# Autodesk Inventor assembly: FE-00035-02
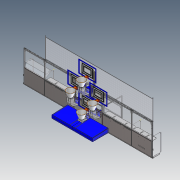
[picture p0: Inventor's stored thumbnail of the model, 180x180]
Saved by Autodesk Inventor 2012 (Build 160160000, 160)
## iProperties
Created: 2010-11-28
Part Number: FE-00035-02
Document SubType Name: Assembly
Designer: dfoster
Description: End Panel Sub-Assembly
Title: End Panel Sub-Assembly
Author: dfoster
## Documents named in this file (24)
- C:\Data Folder\FRC 2012 Field\Components\FE-00035-02.iam
- C:\Data Folder\FRC 2012 Field\Components\FE-00004.iam
- C:\Data Folder\FRC 2012 Field\Components\FE-00001.iam
- C:\Data Folder\FRC 2012 Field\Components\FE-00002-11.iam
- C:\Data Folder\FRC 2012 Field\Components\FE-00002-12.iam
- C:\Data Folder\FRC 2012 Field\Components\FE-00012.ipt
- C:\Data Folder\FRC 2012 Field\Components\GE-11041r.iam
- C:\Data Folder\FRC 2012 Field\Components\GE-11041L.iam
- C:\Data Folder\FRC 2012 Field\Components\GE-09031.iam
- C:\Data Folder\FRC 2012 Field\Components\FE-00007.iam
- C:\Data Folder\FRC 2012 Field\Components\GE-12096.iam
- C:\Data Folder\FRC 2012 Field\Components\GE-12051.ipt
- C:\Data Folder\FRC 2012 Field\Components\GE-12055.ipt
- C:\Data Folder\FRC 2012 Field\Components\GE-12053.iam
- C:\Data Folder\FRC 2012 Field\Components\GE-12057.iam
- C:\Data Folder\FRC 2012 Field\Components\GE-12057_left.iam
- C:\Data Folder\FRC 2012 Field\Components\GE-12056.ipt
- C:\Data Folder\FRC 2012 Field\Components\GE-12078.iam
- C:\Data Folder\FRC 2012 Field\Components\GE-12091.iam
- C:\Data Folder\FRC 2012 Field\Components\GE-12060.ipt
- C:\Data Folder\FRC 2012 Field\Components\GE-12104.ipt
- C:\Data Folder\FRC 2012 Field\Components\HW-00005.0005.ipt
- C:\Data Folder\FRC 2012 Field\Components\HW-00063.ipt
- C:\Data Folder\FRC 2012 Field\Components\HW-00002.ipt
## Components (38 placed, 23 different names)
1. GE-09031:1 [sub-assembly] — Flush:31, Flush:32, Tangent:10, Tangent:15
2. GE-09031:2 [sub-assembly] — Flush:29, Flush:30, Tangent:9, Tangent:16
3. GE-11041r:1 [sub-assembly] — Flush:17, Flush:18, Flush:21, Flush:22, Mate:12, Mate:23, Mate:28, Mate:30, Mate:31, Flush:44
4. GE-11041L:1 [sub-assembly] — Flush:19, Flush:20, Flush:23, Flush:24, Mate:13, Mate:26, Mate:48, Mate:49, Flush:56
5. FE-00002-11:1 [sub-assembly] — Flush:21, Flush:22, Mate:12, Tangent:15, Mate:34, Mate:35, Flush:46, Tangent:19
6. FE-00012:3 — Mate:20, Mate:21, Flush:37, Flush:43, Mate:29
7. FE-00012:1 — Mate:15, Mate:16, Flush:33, Flush:41, Flush:42, Mate:27
8. FE-00002-12:1 [sub-assembly] — Flush:23, Flush:24, Mate:13, Tangent:16
9. FE-00001:3 [sub-assembly] — Mate:7, Flush:13, Flush:14, Flush:17, Tangent:10, Tangent:14, Mate:23, Mate:24
10. FE-00001:4 [sub-assembly] — Flush:9, Mate:5, Flush:10, Flush:19, Tangent:3, Mate:14, Tangent:6, Tangent:9, Mate:26, Mate:36, Mate:37, Flush:47, Tangent:20
11. FE-00004:3 [sub-assembly] — Mate:7, Flush:13, Flush:14, Flush:18, Mate:20, Mate:21, Flush:35, Flush:36, Mate:22, Flush:37
12. FE-00004:2 [sub-assembly] — Flush:9, Mate:5, Flush:10, Flush:20, Mate:15, Mate:16, Flush:33, Flush:38, Mate:25, Flush:39
13. FE-00007:1 [sub-assembly] — Tangent:3, Mate:14, Tangent:6, Flush:29, Flush:30, Flush:40
14. FE-00007:3 [sub-assembly] — Flush:31, Flush:32, Tangent:14, Tangent:17, Mate:24, Flush:40
15. GE-12096:1 [sub-assembly] — Flush:34, Flush:35, Flush:36, Mate:22, Tangent:17, Flush:38, Mate:25, Flush:39, Mate:43, Mate:44, Mate:45, Mate:46, Mate:47, Insert:1, Insert:2, Insert:3, Insert:4
16. GE-12051:1 — Flush:41, Flush:42, Mate:27
17. GE-12055:1 — Flush:43, Mate:28, Mate:29
18. GE-12053:1 [sub-assembly] — Mate:30, Mate:31, Flush:44, Insert:5, Insert:6, Mate:52, Mate:53
19. GE-12060:1 — Mate:48, Mate:49, Flush:56
20. GE-12057:1 [sub-assembly] — Mate:36, Mate:37, Flush:47, Mate:39
21. GE-12057_left:1 [sub-assembly] — Mate:34, Mate:35, Flush:46, Mate:38
22. GE-12056:1 — Mate:38, Tangent:19
23. GE-12056:2 — Mate:39, Tangent:20
24. GE-12104:1
25. GE-12078:1 [sub-assembly] — Mate:43, Mate:44, Flush:55
26. GE-12091:1 [sub-assembly] — Flush:55, Mate:45, Mate:46, Mate:47
27. HW-00005.0005:1 — Insert:4
28. HW-00005.0005:2 — Insert:3
29. HW-00005.0005:3 — Insert:2
30. HW-00005.0005:4 — Insert:1
31. HW-00063:1 — Insert:5, Mate:50
32. HW-00063:2 — Insert:6, Mate:51
33. HW-00002:1 — Mate:50, Mate:52
34. HW-00002:2 — Mate:51, Mate:53
35. HW-00063:3
36. HW-00063:4
37. HW-00002:3
38. HW-00002:4
## Component patterns: (2 elements, first: HW-00063:1 + HW-00063:2 + HW-00002:1 + HW-00002:2)
## Relationships (88: Mate 39, Flush 33, Tangent 10, Insert 6)
- Flush:9: FE-00001:4 ↔ FE-00004:2
- Mate:5 (3.175 mm): FE-00001:4 ↔ FE-00004:2
- Flush:10: FE-00001:4 ↔ FE-00004:2
- Mate:7 (3.175 mm): FE-00001:3 ↔ FE-00004:3
- Flush:13: FE-00001:3 ↔ FE-00004:3
- Flush:14: FE-00001:3 ↔ FE-00004:3
- Flush:17: GE-11041r:1 ↔ FE-00001:3
- Flush:18: GE-11041r:1 ↔ FE-00004:3
- Flush:19: GE-11041L:1 ↔ FE-00001:4
- Flush:20: GE-11041L:1 ↔ FE-00004:2
- Flush:21: GE-11041r:1 ↔ FE-00002-11:1
- Flush:22: GE-11041r:1 ↔ FE-00002-11:1
- Mate:12 (22.225 mm): GE-11041r:1 ↔ FE-00002-11:1
- Flush:23: GE-11041L:1 ↔ FE-00002-12:1
- Flush:24: GE-11041L:1 ↔ FE-00002-12:1
- Mate:13 (22.225 mm): GE-11041L:1 ↔ FE-00002-12:1
- Tangent:3 (0.7874 mm): FE-00001:4 ↔ FE-00007:1
- Mate:14: FE-00001:4 ↔ FE-00007:1
- Tangent:6: FE-00001:4 ↔ FE-00007:1
- Flush:29: GE-09031:2 ↔ FE-00007:1
- Flush:30: GE-09031:2 ↔ FE-00007:1
- Tangent:9: GE-09031:2 ↔ FE-00001:4
- Flush:31: GE-09031:1 ↔ FE-00007:3
- Flush:32: GE-09031:1 ↔ FE-00007:3
- Tangent:10: GE-09031:1 ↔ FE-00001:3
- Mate:15: FE-00012:1 ↔ FE-00004:2
- Mate:16: FE-00012:1 ↔ FE-00004:2
- Flush:33: FE-00012:1 ↔ FE-00004:2
- Mate:20: FE-00012:3 ↔ FE-00004:3
- Mate:21: FE-00012:3 ↔ FE-00004:3
- Tangent:14 (0.7874 mm): FE-00001:3 ↔ FE-00007:3
- Tangent:15: GE-09031:1 ↔ FE-00002-11:1
- Tangent:16: GE-09031:2 ↔ FE-00002-12:1
- Flush:34: GE-12096:1
- Flush:35: FE-00004:3 ↔ GE-12096:1
- Flush:36: FE-00004:3 ↔ GE-12096:1
- Mate:22 (3.175 mm): FE-00004:3 ↔ GE-12096:1
- Mate:23 (3.175 mm): GE-11041r:1 ↔ FE-00001:3
- Flush:37: FE-00012:3 ↔ FE-00004:3
- Tangent:17: FE-00007:3 ↔ GE-12096:1
- Mate:24: FE-00001:3 ↔ FE-00007:3
- Flush:38: FE-00004:2 ↔ GE-12096:1
- Mate:25: FE-00004:2 ↔ GE-12096:1
- Flush:39: FE-00004:2 ↔ GE-12096:1
- Mate:26: GE-11041L:1 ↔ FE-00001:4
- Flush:40: FE-00007:1 ↔ FE-00007:3
- Flush:41: FE-00012:1 ↔ GE-12051:1
- Flush:42: FE-00012:1 ↔ GE-12051:1
- Mate:27 (9.525 mm): FE-00012:1 ↔ GE-12051:1
- Flush:43: FE-00012:3 ↔ GE-12055:1
- Mate:28: GE-11041r:1 ↔ GE-12055:1
- Mate:29 (12.7 mm): FE-00012:3 ↔ GE-12055:1
- Mate:30: GE-11041r:1 ↔ GE-12053:1
- Mate:31 (3.175 mm): GE-11041r:1 ↔ GE-12053:1
- Flush:44: GE-11041r:1 ↔ GE-12053:1
- Mate:34: FE-00002-11:1 ↔ GE-12057_left:1
- Mate:35: FE-00002-11:1 ↔ GE-12057_left:1
- Flush:46 (-3.175 mm): FE-00002-11:1 ↔ GE-12057_left:1
- Mate:36: FE-00001:4 ↔ GE-12057:1
- Mate:37: FE-00001:4 ↔ GE-12057:1
- Flush:47 (-3.175 mm): FE-00001:4 ↔ GE-12057:1
- Mate:38: GE-12057_left:1 ↔ GE-12056:1
- Tangent:19: FE-00002-11:1 ↔ GE-12056:1
- Mate:39: GE-12057:1 ↔ GE-12056:2
- Tangent:20: FE-00001:4 ↔ GE-12056:2
- [Mate]: GE-12056:1 ↔ GE-12104:1
- [Mate]: FE-00007:3 ↔ GE-12104:1
- [Mate] (-3.175 mm): GE-12056:1 ↔ GE-12104:1
- [Flush]: GE-12096:1 ↔ GE-12078:1
- Mate:43: GE-12096:1 ↔ GE-12078:1
- Mate:44 (30.1625 mm): GE-12096:1 ↔ GE-12078:1
- Flush:55: GE-12078:1 ↔ GE-12091:1
- Mate:45: GE-12096:1 ↔ GE-12091:1
- Mate:46 (1.5875 mm): GE-12096:1 ↔ GE-12091:1
- Mate:47: GE-12096:1 ↔ GE-12091:1
- Mate:48: GE-11041L:1 ↔ GE-12060:1
- Mate:49: GE-11041L:1 ↔ GE-12060:1
- Flush:56: GE-11041L:1 ↔ GE-12060:1
- Insert:1: GE-12096:1 ↔ HW-00005.0005:4
- Insert:2: GE-12096:1 ↔ HW-00005.0005:3
- Insert:3: GE-12096:1 ↔ HW-00005.0005:2
- Insert:4: GE-12096:1 ↔ HW-00005.0005:1
- Insert:5: GE-12053:1 ↔ HW-00063:1
- Insert:6: GE-12053:1 ↔ HW-00063:2
- Mate:50: HW-00063:1 ↔ HW-00002:1
- Mate:51: HW-00063:2 ↔ HW-00002:2
- Mate:52: GE-12053:1 ↔ HW-00002:1
- Mate:53: GE-12053:1 ↔ HW-00002:2
